# Autodesk Inventor assembly: TeslaCoil
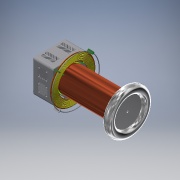
[picture p0: Inventor's stored thumbnail of the model, 180x180]
Saved by Autodesk Inventor 2019 (Build 230136000, 136)
## iProperties
Created: 2021-01-17
Part Number: TeslaCoil
Material: Типовые
Document SubType Name: Assembly
Designer: Dazer
Author: Dazer
## Documents named in this file (13)
- C:\Users\Dazer\Documents\GitHub\Tesla_coil_V1\3dModels\TeslaCoil.iam
- C:\Users\Dazer\Documents\GitHub\Tesla_coil_V1\3dModels\TopBox.ipt
- C:\Users\Dazer\Documents\GitHub\Tesla_coil_V1\3dModels\RackeSecondary.ipt
- C:\Users\Dazer\Documents\GitHub\Tesla_coil_V1\3dModels\PrimaryTab.ipt
- C:\Users\Dazer\Documents\GitHub\Tesla_coil_V1\3dModels\PrimaryCoil.ipt
- C:\Users\Dazer\Documents\GitHub\Tesla_coil_V1\3dModels\Cap.ipt
- C:\Users\Dazer\Documents\GitHub\Tesla_coil_V1\3dModels\Coil.ipt
- C:\Users\Dazer\Documents\GitHub\Tesla_coil_V1\3dModels\Toroid.ipt
- C:\Users\Dazer\Documents\GitHub\Tesla_coil_V1\3dModels\Staicring.ipt
- C:\Users\Dazer\Documents\GitHub\Tesla_coil_V1\3dModels\SecindaryCap.ipt
- C:\Users\Dazer\Documents\GitHub\Tesla_coil_V1\3dModels\BottomBox.ipt
- C:\Users\Dazer\Documents\GitHub\Tesla_coil_V1\3dModels\Legs.ipt
- C:\Users\Dazer\Documents\GitHub\Tesla_coil_V1\3dModels\RackeSecondaryStacring.ipt
## Components (19 placed, 12 different names)
1. TopBox:1 — Совмещение:9, Совмещение:10, Совмещение:15, Совмещение:16, Совмещение:17, Совмещение:18, Заподлицо:3, Заподлицо:4, Заподлицо:6
2. RackeSecondary:1
3. RackeSecondary:2 — Совмещение:15, Совмещение:16, Заподлицо:1, Заподлицо:2
4. RackeSecondary:3 — Совмещение:17, Совмещение:18
5. PrimaryTab:1
6. PrimaryCoil:1
7. Cap:1 — Совмещение:9, Совмещение:10, Совмещение:11, Совмещение:21
8. Cap:2 — Совмещение:12, Совмещение:13
9. Coil:1 — Совмещение:11, Совмещение:12
10. Toroid:1 — Совмещение:13, Совмещение:14
11. Toroid:2 — Совмещение:14
12. Staicring:1 — Заподлицо:1, Заподлицо:2, Совмещение:21
13. SecindaryCap:1 — Заподлицо:3
14. BottomBox:1 — Заподлицо:4, Заподлицо:5, Совмещение:22, Совмещение:23, Совмещение:24
15. Legs:1 — Заподлицо:5
16. Legs:2 — Совмещение:22
17. Legs:3 — Совмещение:24
18. Legs:4 — Совмещение:23
19. RackeSecondaryStacring:1 — Заподлицо:7
## Relationships (21: Mate 14, Flush 7)
- Совмещение:9 [Mate]: TopBox:1 ↔ Cap:1
- Совмещение:10 [Mate]: TopBox:1 ↔ Cap:1
- Совмещение:11 [Mate]: Cap:1 ↔ Coil:1
- Совмещение:12 [Mate]: Cap:2 ↔ Coil:1
- Совмещение:13 [Mate]: Cap:2 ↔ Toroid:1
- Совмещение:14 [Mate]: Toroid:1 ↔ Toroid:2
- Совмещение:15 [Mate]: TopBox:1 ↔ RackeSecondary:2
- Совмещение:16 [Mate]: TopBox:1 ↔ RackeSecondary:2
- Совмещение:17 [Mate]: TopBox:1 ↔ RackeSecondary:3
- Совмещение:18 [Mate]: TopBox:1 ↔ RackeSecondary:3
- Заподлицо:1 [Flush]: RackeSecondary:2 ↔ Staicring:1
- Заподлицо:2 [Flush] (-1.5 mm): RackeSecondary:2 ↔ Staicring:1
- Совмещение:21 [Mate]: Cap:1 ↔ Staicring:1
- Заподлицо:3 [Flush]: TopBox:1 ↔ SecindaryCap:1
- Заподлицо:4 [Flush]: TopBox:1 ↔ BottomBox:1
- Заподлицо:5 [Flush]: BottomBox:1 ↔ Legs:1
- Совмещение:22 [Mate]: BottomBox:1 ↔ Legs:2
- Совмещение:23 [Mate]: BottomBox:1 ↔ Legs:4
- Совмещение:24 [Mate]: BottomBox:1 ↔ Legs:3
- Заподлицо:6 [Flush] (0.2 mm): TopBox:1
- Заподлицо:7 [Flush]: RackeSecondaryStacring:1
